# Autodesk Inventor assembly: Maquete Completa_999
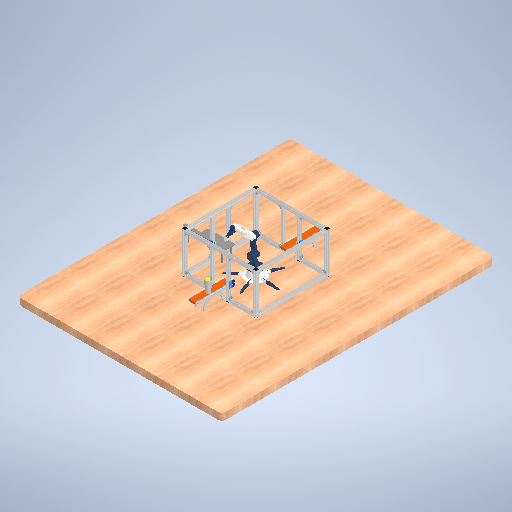
[picture p0: Inventor's stored thumbnail of the model, 512x512]
Saved by Autodesk Inventor 2026 (Build 300175000, 175)
## iProperties
Created: 2024-04-02
Part Number: Maquete Completa_999
Document SubType Name: Assembly
Designer: Gustavo Sousa
Sending System: Autodesk Translation Framework v12.20.1.177
Preprocessor: ST-DEVELOPER v20
Title: Brazo Robtivo 2023 v144.step
## Documents named in this file (40)
- C:\Users\carlo\Documents\Projeto - Braco Robotico\Design\Maquete Completa\Maquete Completa_999.iam
- C:\Users\carlo\Documents\Projeto - Braco Robotico\Design\Maquete Completa\Brazo Robótivo 2023 v144\Engranaje1.ipt
- C:\Users\carlo\Documents\Projeto - Braco Robotico\Design\Maquete Completa\Brazo Robótivo 2023 v144\Engranaje2.ipt
- C:\Users\carlo\Documents\Projeto - Braco Robotico\Design\Maquete Completa\Brazo Robótivo 2023 v144\Barra2.ipt
- C:\Users\carlo\Documents\Projeto - Braco Robotico\Design\Maquete Completa\Brazo Robótivo 2023 v144\Barra1.ipt
- C:\Users\carlo\Documents\Projeto - Braco Robotico\Design\Maquete Completa\Brazo Robótivo 2023 v144\Pinza1.ipt
- C:\Users\carlo\Documents\Projeto - Braco Robotico\Design\Maquete Completa\Brazo Robótivo 2023 v144\Pinza2.ipt
- C:\Users\carlo\Documents\Projeto - Braco Robotico\Design\Maquete Completa\Brazo Robótivo 2023 v144\Base de la garra.ipt
- C:\Users\carlo\Documents\Projeto - Braco Robotico\Design\Maquete Completa\Brazo Robótivo 2023 v144\Base (1) (1).ipt
- C:\Users\carlo\Documents\Projeto - Braco Robotico\Design\Maquete Completa\Brazo Robótivo 2023 v144\Antebrazo (4).ipt
- C:\Users\carlo\Documents\Projeto - Braco Robotico\Design\Maquete Completa\Brazo Robótivo 2023 v144\Muñeca.ipt
- C:\Users\carlo\Documents\Projeto - Braco Robotico\Design\Maquete Completa\Brazo Robótivo 2023 v144\Eje Central.ipt
- C:\Users\carlo\Documents\Projeto - Braco Robotico\Design\Maquete Completa\Brazo Robótivo 2023 v144\Tapa Eje.ipt
- C:\Users\carlo\Documents\Projeto - Braco Robotico\Design\Maquete Completa\Brazo Robótivo 2023 v144\Tapa Base.ipt
- C:\Users\carlo\Documents\Projeto - Braco Robotico\Design\Maquete Completa\Brazo Robótivo 2023 v144\Brazo.ipt
- C:\Users\carlo\Documents\Projeto - Braco Robotico\Design\Maquete Completa\Brazo Robótivo 2023 v144\Tapa garra.ipt
- C:\Users\carlo\Documents\Projeto - Braco Robotico\Design\Maquete Completa\Brazo Robótivo 2023 v144\Pata1.ipt
- C:\Users\carlo\Documents\Projeto - Braco Robotico\Design\Maquete Completa\Brazo Robótivo 2023 v144\Pata2.ipt
- C:\Users\carlo\Documents\Projeto - Braco Robotico\Design\Maquete Completa\Brazo Robótivo 2023 v144\Pata3.ipt
- C:\Users\carlo\Documents\Projeto - Braco Robotico\Design\Maquete Completa\Brazo Robótivo 2023 v144\Pata4.ipt
- C:\Users\carlo\Documents\Projeto - Braco Robotico\Design\Maquete Completa\Brazo Robótivo 2023 v144\Pata5.ipt
- C:\Users\carlo\Documents\Projeto - Braco Robotico\Design\Maquete Completa\Brazo Robótivo 2023 v144\Seguro de servomotor.ipt
- C:\Users\carlo\Documents\Projeto - Braco Robotico\Design\Maquete Completa\maquete_001_001.ipt
- C:\Users\carlo\Documents\Projeto - Braco Robotico\Design\Maquete Completa\perfil_20x20_001.ipt
- C:\Users\carlo\Documents\Projeto - Braco Robotico\Design\Maquete Completa\perfil_20x20_002.ipt
- C:\Users\carlo\Documents\Projeto - Braco Robotico\Design\Maquete Completa\perfil_20x20_003.ipt
- C:\Users\carlo\Documents\Projeto - Braco Robotico\Design\Maquete Completa\perfil_20x20_004.ipt
- C:\Users\carlo\Documents\Projeto - Braco Robotico\Design\Maquete Completa\tampa_001_001.ipt
- C:\Users\carlo\Documents\Projeto - Braco Robotico\Design\Maquete Completa\BPN06M4\BPN06M4\BPN06M4.ipt
- C:\Users\carlo\Documents\Projeto - Braco Robotico\Design\Maquete Completa\CBR2020\CBR2020\CBR2020.ipt
- C:\Users\carlo\Documents\Inventor\Content Center Files\R2026\en-US\BS 4183(4)\BS 4183 - M4 x 8(1) III.ipt
- C:\Users\carlo\Documents\Projeto - Braco Robotico\Design\Maquete Completa\Conveyor_001_001.ipt
- C:\Users\carlo\Documents\Projeto - Braco Robotico\Design\Maquete Completa\Conveyor_002_001.ipt
- C:\Users\carlo\Documents\Projeto - Braco Robotico\Design\Maquete Completa\Conveyor_003_001.ipt
- C:\Users\carlo\Documents\Projeto - Braco Robotico\Design\Maquete Completa\HCSR04 Ultrasonic Sensor\HCSR04 Ultrasonic Sensor\HCSR04 Ultrasonic Sensor.ipt
- C:\Users\carlo\Documents\Projeto - Braco Robotico\Design\Maquete Completa\suporte_ultrassonico_001.ipt
- C:\Users\carlo\Documents\Inventor\Content Center Files\R2026\en-US\BS 4183(1)\BS 4183 - M1,6(1).ipt
- C:\Users\carlo\Documents\Inventor\Content Center Files\R2026\en-US\CSN 02 1131  A\CSN 02 1131 - M1,6 x 6A.ipt
- C:\Users\carlo\Documents\Projeto - Braco Robotico\Design\Maquete Completa\mesa_001.ipt
- C:\Users\carlo\Documents\Projeto - Braco Robotico\Design\Maquete Completa\copo_001.ipt
## Components (249 placed, 39 different names)
1. maquete_001_001:1 — Flush:4, Flush:5, Mate:28, Flush:8, Flush:25, Mate:73, Mate:92, Flush:66, Mate:102, Flush:68, Mate:115, Flush:79, Mate:165
2. mesa_001:1 — Flush:79, Mate:165, Mate:166
3. copo_001:1
4. Engranaje1:1 — Mate:24, Mate:25, Insert:10
5. Engranaje2:1 — Mate:22, Mate:23, Insert:11
6. Barra2:1 — Insert:8, Mate:27
7. Barra1:1 — Insert:9, Mate:26
8. Pinza1:1 — Insert:10, Mate:26
9. Pinza2:1 — Insert:11, Mate:27
10. Base de la garra:1 — Insert:6, Mate:21, Insert:8, Insert:9, Insert:12
11. Base (1) (1):1 — Mate:7, Mate:8, Mate:9, Mate:10, Mate:11, Mate:12, Mate:13, Mate:14, Mate:15, Mate:16, Mate:17, Mate:18, Insert:1, Flush:1, Flush:2, Flush:3, Flush:4, Mate:28
12. Antebrazo (4):1 — Insert:2, Insert:4
13. Muñeca:1 — Insert:5, Insert:12
14. Eje Central:1 — Insert:1, Mate:19, Mate:20, Insert:2
15. Tapa Eje:1 — Mate:19, Mate:20
16. Tapa Base:1 — Mate:17, Mate:18
17. Brazo:1 — Insert:3, Insert:4, Insert:5
18. Tapa garra:1 — Insert:6, Mate:21, Mate:22, Mate:23, Mate:24, Mate:25
19. Pata1:1 — Mate:9, Mate:10
20. Pata2:1 — Mate:11, Mate:12
21. Pata3:1 — Mate:15, Mate:16
22. Pata4:1 — Mate:13, Mate:14
23. Pata5:1 — Mate:7, Mate:8
24. Seguro de servomotor:1 — Insert:3
25. perfil_20x20_001:4 — Flush:6, Mate:29, Flush:7, Flush:8, Flush:9, Mate:30, Flush:10, Flush:29, Flush:62, Mate:75, Flush:63, Flush:65, Mate:77
26. perfil_20x20_002:4 — Flush:6, Mate:29, Flush:7, Flush:11, Flush:26, Flush:27, Mate:37, Flush:28, Mate:49, Flush:51, Flush:52, Mate:50, Mate:67, Flush:60, Mate:68, Mate:74, Mate:76
27. perfil_20x20_002:5 — Flush:9, Mate:30, Flush:10, Mate:31, Flush:12, Flush:13, Mate:32, Flush:14, Flush:15, Mate:33, Flush:16, Mate:47, Flush:49, Mate:48, Mate:61, Flush:58, Mate:62
28. perfil_20x20_001:5 — Flush:11, Mate:31, Flush:12, Symmetry:3, Mate:41, Flush:49, Flush:50, Flush:51
29. perfil_20x20_001:6 — Flush:13, Mate:32, Flush:14, Flush:19, Mate:35, Flush:20, Flush:25, Flush:39, Flush:74
30. perfil_20x20_003:1 — Flush:15, Mate:33, Flush:16, Flush:17, Mate:34, Flush:18, Flush:30
31. perfil_20x20_004:1 — Flush:17, Mate:34, Flush:18, Flush:24, Symmetry:1, Mate:63, Flush:59, Mate:64, Flush:73, Mate:127, Mate:128, Mate:129
32. perfil_20x20_002:6 — Flush:19, Mate:35, Flush:20, Flush:21, Flush:22, Mate:36, Flush:40, Mate:42, Mate:45, Flush:48, Mate:46, Mate:53, Flush:54, Mate:54
33. perfil_20x20_003:2 — Flush:21, Flush:22, Mate:36, Flush:23, Flush:41
34. perfil_20x20_004:2 — Flush:23, Flush:24, Symmetry:1, Flush:42, Mate:65, Mate:66
35. perfil_20x20_001:7 — Flush:26, Flush:27, Mate:37, Flush:33, Mate:39, Flush:34
36. perfil_20x20_003:3 — Flush:28, Flush:29, Flush:30, Flush:31, Flush:32, Mate:38
37. perfil_20x20_004:3 — Flush:31, Flush:32, Mate:38, Symmetry:2, Flush:38, Mate:71, Flush:61, Mate:72, Flush:70, Mate:106, Flush:71, Mate:107, Mate:110
38. perfil_20x20_002:7 — Flush:33, Mate:39, Flush:34, Flush:35, Mate:40, Flush:36, Flush:44, Mate:44, Flush:45, Mate:51, Flush:53, Mate:52, Mate:59, Flush:57, Mate:60, Flush:76, Flush:77
39. perfil_20x20_003:4 — Flush:35, Mate:40, Flush:36, Flush:37
40. perfil_20x20_004:4 — Flush:37, Symmetry:2, Flush:38, Mate:69, Mate:70
41. perfil_20x20_001:8 — Flush:39, Symmetry:3, Mate:41
42. perfil_20x20_003:5 — Flush:40, Flush:41, Mate:42, Mate:43, Flush:43, Symmetry:4
43. perfil_20x20_004:5 — Flush:42, Mate:43, Flush:43, Flush:47, Symmetry:5, Mate:55, Flush:55, Mate:56
44. perfil_20x20_003:6 — Symmetry:4, Flush:44, Mate:44, Flush:45, Flush:46
45. perfil_20x20_004:6 — Flush:46, Flush:47, Symmetry:5, Mate:57, Flush:56, Mate:58, Mate:140, Mate:141, Mate:142, Mate:166
46. tampa_001_001:1 — Mate:45, Flush:48, Mate:46
47. tampa_001_001:2 — Mate:47, Flush:50, Mate:48
48. tampa_001_001:3 — Mate:49, Flush:52, Mate:50
49. tampa_001_001:4 — Mate:51, Flush:53, Mate:52
50. tampa_001_001:5 — Mate:53, Flush:54, Mate:54
51. tampa_001_001:6 — Mate:55, Flush:55, Mate:56
52. tampa_001_001:7 — Mate:57, Flush:56, Mate:58
53. tampa_001_001:8 — Mate:59, Flush:57, Mate:60
54. tampa_001_001:9 — Mate:61, Flush:58, Mate:62
55. tampa_001_001:10 — Mate:67, Flush:60, Mate:68
56. tampa_001_001:11 — Mate:65, Mate:66
57. tampa_001_001:12 — Mate:63, Flush:59, Mate:64
58. tampa_001_001:13 — Mate:71, Flush:61, Mate:72, Mate:73
59. tampa_001_001:14 — Mate:69, Mate:70
60. CBR2020:2
61. BPN06M4:63
62. BPN06M4:64
63. BS 4183 Specification for machine screws and machine screw nuts. Metric series - Metric M4 x 8:63
64. BS 4183 Specification for machine screws and machine screw nuts. Metric series - Metric M4 x 8:64
65. CBR2020:14
66. BPN06M4:87
67. BPN06M4:88
68. BS 4183 Specification for machine screws and machine screw nuts. Metric series - Metric M4 x 8:87
69. BS 4183 Specification for machine screws and machine screw nuts. Metric series - Metric M4 x 8:88
70. CBR2020:15
71. BPN06M4:89
72. BPN06M4:90
73. BS 4183 Specification for machine screws and machine screw nuts. Metric series - Metric M4 x 8:89
74. BS 4183 Specification for machine screws and machine screw nuts. Metric series - Metric M4 x 8:90
75. CBR2020:16
76. BPN06M4:91
77. BPN06M4:92
78. BS 4183 Specification for machine screws and machine screw nuts. Metric series - Metric M4 x 8:91
79. BS 4183 Specification for machine screws and machine screw nuts. Metric series - Metric M4 x 8:92
80. CBR2020:17
81. BPN06M4:93
82. BPN06M4:94
83. BS 4183 Specification for machine screws and machine screw nuts. Metric series - Metric M4 x 8:93
84. BS 4183 Specification for machine screws and machine screw nuts. Metric series - Metric M4 x 8:94
85. CBR2020:18
86. BPN06M4:95
87. BPN06M4:96
88. BS 4183 Specification for machine screws and machine screw nuts. Metric series - Metric M4 x 8:95
89. BS 4183 Specification for machine screws and machine screw nuts. Metric series - Metric M4 x 8:96
90. CBR2020:19
91. BPN06M4:97
92. BPN06M4:98
93. BS 4183 Specification for machine screws and machine screw nuts. Metric series - Metric M4 x 8:97
94. BS 4183 Specification for machine screws and machine screw nuts. Metric series - Metric M4 x 8:98
95. CBR2020:20
96. BPN06M4:99
97. BPN06M4:100
98. BS 4183 Specification for machine screws and machine screw nuts. Metric series - Metric M4 x 8:99
99. BS 4183 Specification for machine screws and machine screw nuts. Metric series - Metric M4 x 8:100
100. CBR2020:21
101. BPN06M4:101
102. BPN06M4:102
103. BS 4183 Specification for machine screws and machine screw nuts. Metric series - Metric M4 x 8:101
104. BS 4183 Specification for machine screws and machine screw nuts. Metric series - Metric M4 x 8:102
105. CBR2020:22
106. BPN06M4:103
107. BPN06M4:104
108. BS 4183 Specification for machine screws and machine screw nuts. Metric series - Metric M4 x 8:103
109. BS 4183 Specification for machine screws and machine screw nuts. Metric series - Metric M4 x 8:104
110. CBR2020:23
111. BPN06M4:105
112. BPN06M4:106
113. BS 4183 Specification for machine screws and machine screw nuts. Metric series - Metric M4 x 8:105
114. BS 4183 Specification for machine screws and machine screw nuts. Metric series - Metric M4 x 8:106
115. CBR2020:24
116. BPN06M4:107
117. BPN06M4:108
118. BS 4183 Specification for machine screws and machine screw nuts. Metric series - Metric M4 x 8:107
119. BS 4183 Specification for machine screws and machine screw nuts. Metric series - Metric M4 x 8:108
120. CBR2020:25
121. BPN06M4:109
122. BPN06M4:110
123. BS 4183 Specification for machine screws and machine screw nuts. Metric series - Metric M4 x 8:109
124. BS 4183 Specification for machine screws and machine screw nuts. Metric series - Metric M4 x 8:110
125. CBR2020:26
126. BPN06M4:111
127. BPN06M4:112
128. BS 4183 Specification for machine screws and machine screw nuts. Metric series - Metric M4 x 8:111
129. BS 4183 Specification for machine screws and machine screw nuts. Metric series - Metric M4 x 8:112
130. CBR2020:27
131. BPN06M4:113
132. BPN06M4:114
133. BS 4183 Specification for machine screws and machine screw nuts. Metric series - Metric M4 x 8:113
134. BS 4183 Specification for machine screws and machine screw nuts. Metric series - Metric M4 x 8:114
135. CBR2020:28
136. BPN06M4:115
137. BPN06M4:116
138. BS 4183 Specification for machine screws and machine screw nuts. Metric series - Metric M4 x 8:115
139. BS 4183 Specification for machine screws and machine screw nuts. Metric series - Metric M4 x 8:116
140. CBR2020:3
141. BPN06M4:65
142. BPN06M4:66
143. BS 4183 Specification for machine screws and machine screw nuts. Metric series - Metric M4 x 8:65
144. BS 4183 Specification for machine screws and machine screw nuts. Metric series - Metric M4 x 8:66
145. CBR2020:4
146. BPN06M4:67
147. BPN06M4:68
148. BS 4183 Specification for machine screws and machine screw nuts. Metric series - Metric M4 x 8:67
149. BS 4183 Specification for machine screws and machine screw nuts. Metric series - Metric M4 x 8:68
150. CBR2020:5
151. BPN06M4:69
152. BPN06M4:70
153. BS 4183 Specification for machine screws and machine screw nuts. Metric series - Metric M4 x 8:69
154. BS 4183 Specification for machine screws and machine screw nuts. Metric series - Metric M4 x 8:70
155. CBR2020:6
156. BPN06M4:71
157. BPN06M4:72
158. BS 4183 Specification for machine screws and machine screw nuts. Metric series - Metric M4 x 8:71
159. BS 4183 Specification for machine screws and machine screw nuts. Metric series - Metric M4 x 8:72
160. CBR2020:7
161. BPN06M4:73
162. BPN06M4:74
163. BS 4183 Specification for machine screws and machine screw nuts. Metric series - Metric M4 x 8:73
164. BS 4183 Specification for machine screws and machine screw nuts. Metric series - Metric M4 x 8:74
165. CBR2020:8
166. BPN06M4:75
167. BPN06M4:76
168. BS 4183 Specification for machine screws and machine screw nuts. Metric series - Metric M4 x 8:75
169. BS 4183 Specification for machine screws and machine screw nuts. Metric series - Metric M4 x 8:76
170. CBR2020:9
171. BPN06M4:77
172. BPN06M4:78
173. BS 4183 Specification for machine screws and machine screw nuts. Metric series - Metric M4 x 8:77
174. BS 4183 Specification for machine screws and machine screw nuts. Metric series - Metric M4 x 8:78
175. CBR2020:10
176. BPN06M4:79
177. BPN06M4:80
178. BS 4183 Specification for machine screws and machine screw nuts. Metric series - Metric M4 x 8:79
179. BS 4183 Specification for machine screws and machine screw nuts. Metric series - Metric M4 x 8:80
180. CBR2020:11
181. BPN06M4:81
182. BPN06M4:82
183. BS 4183 Specification for machine screws and machine screw nuts. Metric series - Metric M4 x 8:81
184. BS 4183 Specification for machine screws and machine screw nuts. Metric series - Metric M4 x 8:82
185. CBR2020:12
186. BPN06M4:83
187. BPN06M4:84
188. BS 4183 Specification for machine screws and machine screw nuts. Metric series - Metric M4 x 8:83
189. BS 4183 Specification for machine screws and machine screw nuts. Metric series - Metric M4 x 8:84
190. CBR2020:13
191. BPN06M4:85
192. BPN06M4:86
193. BS 4183 Specification for machine screws and machine screw nuts. Metric series - Metric M4 x 8:85
194. BS 4183 Specification for machine screws and machine screw nuts. Metric series - Metric M4 x 8:86
195. CBR2020:1 — Flush:62, Mate:74, Mate:75, Flush:64, Mate:78, Mate:80, Mate:82
196. BPN06M4:1 — Flush:65, Mate:77, Mate:78, Mate:81
197. BPN06M4:2 — Flush:63, Mate:76, Flush:64, Mate:79
198. BS 4183 Specification for machine screws and machine screw nuts. Metric series - Metric M4 x 8:1 — Mate:79, Mate:80
199. BS 4183 Specification for machine screws and machine screw nuts. Metric series - Metric M4 x 8:2 — Mate:81, Mate:82
200. Conveyor_002_001:1 — Mate:83, Mate:84, Mate:85, Mate:91
201. Conveyor_002_001:2 — Mate:86, Mate:87, Mate:88, Mate:89
202. Conveyor_003_001:1 — Mate:89, Mate:90, Mate:91
203. Conveyor_001_001:2 — Mate:83, Mate:84, Mate:85, Mate:86, Mate:87, Mate:88, Mate:90, Mate:92, Flush:66, Flush:72
204. Conveyor_001_001:3 — Mate:102, Flush:68, Flush:75
205. Conveyor_002_001:3
206. Conveyor_002_001:4
207. Conveyor_003_001:2
208. suporte_ultrassonico_001:3 — Mate:137, Mate:138, Mate:139, Mate:142, Mate:143, Mate:144, Mate:145, Mate:146, Mate:147, Mate:148, Mate:149, Mate:150, Mate:151, Mate:152, Mate:153, Mate:154, Mate:155, Mate:156
209. HCSR04 Ultrasonic Sensor:3 — Mate:137, Mate:138, Mate:139, Flush:78, Mate:161, Mate:162, Mate:163, Mate:164
210. BPN06M4:61 — Flush:77, Mate:141, Mate:144
211. BPN06M4:62 — Flush:76, Mate:140, Mate:143
212. BS 4183 Specification for machine screws and machine screw nuts. Metric series - Metric M4 x 8:61 — Mate:145, Mate:147
213. BS 4183 Specification for machine screws and machine screw nuts. Metric series - Metric M4 x 8:62 — Mate:146, Mate:148
214. CSN 02 1131 A M1,6 x 6:9 — Mate:149, Mate:154, Mate:157
215. CSN 02 1131 A M1,6 x 6:10 — Mate:152, Mate:156, Mate:160
216. CSN 02 1131 A M1,6 x 6:11 — Mate:151, Mate:155, Mate:159
217. CSN 02 1131 A M1,6 x 6:12 — Mate:150, Mate:153, Mate:158
218. BS 4183 - Metric M1,6:9 — Mate:158, Mate:162
219. BS 4183 - Metric M1,6:10 — Mate:160, Mate:163
220. BS 4183 - Metric M1,6:11 — Mate:159, Mate:164
221. BS 4183 - Metric M1,6:12 — Mate:157, Mate:161
222. suporte_ultrassonico_001:2 — Mate:116, Mate:117, Mate:118, Insert:21, Insert:22, Insert:23, Insert:24, Mate:129, Mate:130, Mate:131, Mate:132, Mate:133, Mate:134, Mate:135
223. HCSR04 Ultrasonic Sensor:2 — Mate:116, Mate:117, Mate:118, Mate:120, Mate:122, Mate:124, Mate:126, Mate:136, Flush:75
224. CSN 02 1131 A M1,6 x 6:5 — Insert:21, Mate:123
225. CSN 02 1131 A M1,6 x 6:6 — Insert:22, Mate:125
226. CSN 02 1131 A M1,6 x 6:7 — Insert:23, Mate:119
227. CSN 02 1131 A M1,6 x 6:8 — Insert:24, Mate:121
228. BS 4183 - Metric M1,6:5 — Mate:119, Mate:120
229. BS 4183 - Metric M1,6:6 — Mate:121, Mate:122
230. BS 4183 - Metric M1,6:7 — Mate:123, Mate:124
231. BS 4183 - Metric M1,6:8 — Mate:125, Mate:126
232. BPN06M4:59 — Flush:74, Mate:128, Mate:131
233. BPN06M4:60 — Flush:73, Mate:127, Mate:130
234. BS 4183 Specification for machine screws and machine screw nuts. Metric series - Metric M4 x 8:59 — Mate:133, Mate:134
235. BS 4183 Specification for machine screws and machine screw nuts. Metric series - Metric M4 x 8:60 — Mate:132, Mate:135
236. BS 4183 - Metric M1,6:1 — Insert:13
237. BS 4183 - Metric M1,6:2 — Insert:14
238. BS 4183 - Metric M1,6:3 — Insert:15
239. BS 4183 - Metric M1,6:4 — Insert:16
240. CSN 02 1131 A M1,6 x 6:2 — Insert:17
241. CSN 02 1131 A M1,6 x 6:3 — Insert:18
242. CSN 02 1131 A M1,6 x 6:1 — Insert:19
243. CSN 02 1131 A M1,6 x 6:4 — Insert:20
244. HCSR04 Ultrasonic Sensor:1 — Mate:103, Mate:104, Mate:105, Insert:13, Insert:14, Insert:15, Insert:16, Flush:72, Mate:136, Flush:78
245. suporte_ultrassonico_001:1 — Mate:103, Mate:104, Mate:105, Mate:108, Mate:109, Mate:110, Mate:112, Mate:114, Mate:115, Insert:17, Insert:18, Insert:19, Insert:20
246. BPN06M4:58 — Flush:70, Mate:106, Mate:109, Mate:111
247. BS 4183 Specification for machine screws and machine screw nuts. Metric series - Metric M4 x 8:57 — Mate:111, Mate:112
248. BS 4183 Specification for machine screws and machine screw nuts. Metric series - Metric M4 x 8:58 — Mate:113, Mate:114
249. BPN06M4:57 — Flush:71, Mate:107, Mate:108, Mate:113
## Relationships (265: Mate 160, Flush 77, Insert 23, Symmetry 5)
- Mate:7: Base (1) (1):1 ↔ Pata5:1
- Mate:8: Base (1) (1):1 ↔ Pata5:1
- Mate:9: Base (1) (1):1 ↔ Pata1:1
- Mate:10: Base (1) (1):1 ↔ Pata1:1
- Mate:11: Base (1) (1):1 ↔ Pata2:1
- Mate:12: Base (1) (1):1 ↔ Pata2:1
- Mate:13: Base (1) (1):1 ↔ Pata4:1
- Mate:14: Base (1) (1):1 ↔ Pata4:1
- Mate:15: Base (1) (1):1 ↔ Pata3:1
- Mate:16: Base (1) (1):1 ↔ Pata3:1
- Mate:17: Base (1) (1):1 ↔ Tapa Base:1
- Mate:18: Base (1) (1):1 ↔ Tapa Base:1
- Insert:1: Base (1) (1):1 ↔ Eje Central:1
- Mate:19: Eje Central:1 ↔ Tapa Eje:1
- Mate:20 (1.05 mm): Eje Central:1 ↔ Tapa Eje:1
- Insert:2: Antebrazo (4):1 ↔ Eje Central:1
- Insert:3: Brazo:1 ↔ Seguro de servomotor:1
- Insert:4: Antebrazo (4):1 ↔ Brazo:1
- Insert:5: Muñeca:1 ↔ Brazo:1
- Insert:6: Base de la garra:1 ↔ Tapa garra:1
- Mate:21: Base de la garra:1 ↔ Tapa garra:1
- Insert:8: Barra2:1 ↔ Base de la garra:1
- Insert:9: Barra1:1 ↔ Base de la garra:1
- Mate:22: Engranaje2:1 ↔ Tapa garra:1
- Mate:23: Engranaje2:1 ↔ Tapa garra:1
- Mate:24: Engranaje1:1 ↔ Tapa garra:1
- Mate:25: Engranaje1:1 ↔ Tapa garra:1
- Insert:10 (0.5 mm): Engranaje1:1 ↔ Pinza1:1
- Mate:26: Barra1:1 ↔ Pinza1:1
- Insert:11: Engranaje2:1 ↔ Pinza2:1
- Mate:27: Barra2:1 ↔ Pinza2:1
- Insert:12: Base de la garra:1 ↔ Muñeca:1
- Flush:1: Base (1) (1):1
- Flush:2: Base (1) (1):1
- Flush:3: Base (1) (1):1
- Flush:4: maquete_001_001:1 ↔ Base (1) (1):1
- Flush:5: maquete_001_001:1
- Mate:28: maquete_001_001:1 ↔ Base (1) (1):1
- Flush:6: perfil_20x20_001:4 ↔ perfil_20x20_002:4
- Mate:29: perfil_20x20_001:4 ↔ perfil_20x20_002:4
- Flush:7: perfil_20x20_001:4 ↔ perfil_20x20_002:4
- Flush:8: maquete_001_001:1 ↔ perfil_20x20_001:4
- Flush:9: perfil_20x20_001:4 ↔ perfil_20x20_002:5
- Mate:30: perfil_20x20_001:4 ↔ perfil_20x20_002:5
- Flush:10: perfil_20x20_001:4 ↔ perfil_20x20_002:5
- Flush:11: perfil_20x20_002:4 ↔ perfil_20x20_001:5
- Mate:31: perfil_20x20_002:5 ↔ perfil_20x20_001:5
- Flush:12: perfil_20x20_002:5 ↔ perfil_20x20_001:5
- Flush:13: perfil_20x20_002:5 ↔ perfil_20x20_001:6
- Mate:32: perfil_20x20_002:5 ↔ perfil_20x20_001:6
- Flush:14: perfil_20x20_002:5 ↔ perfil_20x20_001:6
- Flush:15: perfil_20x20_002:5 ↔ perfil_20x20_003:1
- Mate:33: perfil_20x20_002:5 ↔ perfil_20x20_003:1
- Flush:16: perfil_20x20_002:5 ↔ perfil_20x20_003:1
- Flush:17: perfil_20x20_003:1 ↔ perfil_20x20_004:1
- Mate:34: perfil_20x20_003:1 ↔ perfil_20x20_004:1
- Flush:18: perfil_20x20_003:1 ↔ perfil_20x20_004:1
- Flush:19: perfil_20x20_001:6 ↔ perfil_20x20_002:6
- Mate:35: perfil_20x20_001:6 ↔ perfil_20x20_002:6
- Flush:20: perfil_20x20_001:6 ↔ perfil_20x20_002:6
- Flush:21: perfil_20x20_002:6 ↔ perfil_20x20_003:2
- Flush:22: perfil_20x20_002:6 ↔ perfil_20x20_003:2
- Mate:36: perfil_20x20_002:6 ↔ perfil_20x20_003:2
- Flush:23: perfil_20x20_003:2 ↔ perfil_20x20_004:2
- Flush:24: perfil_20x20_004:1 ↔ perfil_20x20_004:2
- Symmetry:1: perfil_20x20_004:1 ↔ perfil_20x20_004:2
- Flush:25: maquete_001_001:1 ↔ perfil_20x20_001:6
- Flush:26: perfil_20x20_002:4 ↔ perfil_20x20_001:7
- Flush:27: perfil_20x20_002:4 ↔ perfil_20x20_001:7
- Mate:37: perfil_20x20_002:4 ↔ perfil_20x20_001:7
- Flush:28: perfil_20x20_002:4 ↔ perfil_20x20_003:3
- Flush:29: perfil_20x20_001:4 ↔ perfil_20x20_003:3
- Flush:30: perfil_20x20_003:1 ↔ perfil_20x20_003:3
- Flush:31: perfil_20x20_003:3 ↔ perfil_20x20_004:3
- Flush:32: perfil_20x20_003:3 ↔ perfil_20x20_004:3
- Mate:38: perfil_20x20_003:3 ↔ perfil_20x20_004:3
- Flush:33: perfil_20x20_001:7 ↔ perfil_20x20_002:7
- Mate:39: perfil_20x20_001:7 ↔ perfil_20x20_002:7
- Flush:34: perfil_20x20_001:7 ↔ perfil_20x20_002:7
- Flush:35: perfil_20x20_002:7 ↔ perfil_20x20_003:4
- Mate:40: perfil_20x20_002:7 ↔ perfil_20x20_003:4
- Flush:36: perfil_20x20_002:7 ↔ perfil_20x20_003:4
- Flush:37: perfil_20x20_003:4 ↔ perfil_20x20_004:4
- Symmetry:2: perfil_20x20_004:3 ↔ perfil_20x20_004:4
- Flush:38: perfil_20x20_004:3 ↔ perfil_20x20_004:4
- Flush:39: perfil_20x20_001:6 ↔ perfil_20x20_001:8
- Symmetry:3: perfil_20x20_001:5 ↔ perfil_20x20_001:8
- Mate:41: perfil_20x20_001:5 ↔ perfil_20x20_001:8
- Flush:40: perfil_20x20_002:6 ↔ perfil_20x20_003:5
- Flush:41: perfil_20x20_003:2 ↔ perfil_20x20_003:5
- Mate:42: perfil_20x20_002:6 ↔ perfil_20x20_003:5
- Flush:42: perfil_20x20_004:2 ↔ perfil_20x20_004:5
- Mate:43: perfil_20x20_003:5 ↔ perfil_20x20_004:5
- Flush:43: perfil_20x20_003:5 ↔ perfil_20x20_004:5
- Symmetry:4: perfil_20x20_003:5 ↔ perfil_20x20_003:6
- Flush:44: perfil_20x20_002:7 ↔ perfil_20x20_003:6
- Mate:44: perfil_20x20_002:7 ↔ perfil_20x20_003:6
- Flush:45: perfil_20x20_002:7 ↔ perfil_20x20_003:6
- Flush:46: perfil_20x20_003:6 ↔ perfil_20x20_004:6
- Flush:47: perfil_20x20_004:5 ↔ perfil_20x20_004:6
- Symmetry:5: perfil_20x20_004:5 ↔ perfil_20x20_004:6
- Mate:45: perfil_20x20_002:6 ↔ tampa_001_001:1
- Flush:48: perfil_20x20_002:6 ↔ tampa_001_001:1
- Mate:46: perfil_20x20_002:6 ↔ tampa_001_001:1
- Mate:47: perfil_20x20_002:5 ↔ tampa_001_001:2
- Flush:49: perfil_20x20_002:5 ↔ perfil_20x20_001:5
- Flush:50: perfil_20x20_001:5 ↔ tampa_001_001:2
- Mate:48: perfil_20x20_002:5 ↔ tampa_001_001:2
- Mate:49: perfil_20x20_002:4 ↔ tampa_001_001:3
- Flush:51: perfil_20x20_002:4 ↔ perfil_20x20_001:5
- Flush:52: perfil_20x20_002:4 ↔ tampa_001_001:3
- Mate:50: perfil_20x20_002:4 ↔ tampa_001_001:3
- Mate:51: perfil_20x20_002:7 ↔ tampa_001_001:4
- Flush:53: perfil_20x20_002:7 ↔ tampa_001_001:4
- Mate:52: perfil_20x20_002:7 ↔ tampa_001_001:4
- Mate:53: perfil_20x20_002:6 ↔ tampa_001_001:5
- Flush:54: perfil_20x20_002:6 ↔ tampa_001_001:5
- Mate:54: perfil_20x20_002:6 ↔ tampa_001_001:5
- Mate:55: perfil_20x20_004:5 ↔ tampa_001_001:6
- Flush:55: perfil_20x20_004:5 ↔ tampa_001_001:6
- Mate:56: perfil_20x20_004:5 ↔ tampa_001_001:6
- Mate:57: perfil_20x20_004:6 ↔ tampa_001_001:7
- Flush:56: perfil_20x20_004:6 ↔ tampa_001_001:7
- Mate:58: perfil_20x20_004:6 ↔ tampa_001_001:7
- Mate:59: perfil_20x20_002:7 ↔ tampa_001_001:8
- Flush:57: perfil_20x20_002:7 ↔ tampa_001_001:8
- Mate:60: perfil_20x20_002:7 ↔ tampa_001_001:8
- Mate:61: perfil_20x20_002:5 ↔ tampa_001_001:9
- Flush:58: perfil_20x20_002:5 ↔ tampa_001_001:9
- Mate:62: perfil_20x20_002:5 ↔ tampa_001_001:9
- Mate:63: perfil_20x20_004:1 ↔ tampa_001_001:12
- Flush:59: perfil_20x20_004:1 ↔ tampa_001_001:12
- Mate:64: perfil_20x20_004:1 ↔ tampa_001_001:12
- Mate:65: perfil_20x20_004:2 ↔ tampa_001_001:11
- Mate:66: perfil_20x20_004:2 ↔ tampa_001_001:11
- Mate:67: perfil_20x20_002:4 ↔ tampa_001_001:10
- Flush:60: perfil_20x20_002:4 ↔ tampa_001_001:10
- Mate:68: perfil_20x20_002:4 ↔ tampa_001_001:10
- Mate:69: perfil_20x20_004:4 ↔ tampa_001_001:14
- Mate:70: perfil_20x20_004:4 ↔ tampa_001_001:14
- Mate:71: perfil_20x20_004:3 ↔ tampa_001_001:13
- Flush:61: perfil_20x20_004:3 ↔ tampa_001_001:13
- Mate:72: perfil_20x20_004:3 ↔ tampa_001_001:13
- Mate:73: maquete_001_001:1 ↔ tampa_001_001:13
- Flush:62: perfil_20x20_001:4 ↔ CBR2020:1
- Mate:74: perfil_20x20_002:4 ↔ CBR2020:1
- Mate:75: perfil_20x20_001:4 ↔ CBR2020:1
- Flush:63: perfil_20x20_001:4 ↔ BPN06M4:2
- Mate:76: perfil_20x20_002:4 ↔ BPN06M4:2
- Flush:64: CBR2020:1 ↔ BPN06M4:2
- Flush:65: perfil_20x20_001:4 ↔ BPN06M4:1
- Mate:77: perfil_20x20_001:4 ↔ BPN06M4:1
- Mate:78: CBR2020:1 ↔ BPN06M4:1
- Mate:79: BPN06M4:2 ↔ BS 4183 Specification for machine screws and machine screw nuts. Metric series - Metric M4 x 8:1
- Mate:80: CBR2020:1 ↔ BS 4183 Specification for machine screws and machine screw nuts. Metric series - Metric M4 x 8:1
- Mate:81: BPN06M4:1 ↔ BS 4183 Specification for machine screws and machine screw nuts. Metric series - Metric M4 x 8:2
- Mate:82: CBR2020:1 ↔ BS 4183 Specification for machine screws and machine screw nuts. Metric series - Metric M4 x 8:2
- Mate:83: Conveyor_002_001:1 ↔ Conveyor_001_001:2
- Mate:84: Conveyor_002_001:1 ↔ Conveyor_001_001:2
- Mate:85 (1 mm): Conveyor_002_001:1 ↔ Conveyor_001_001:2
- Mate:86: Conveyor_002_001:2 ↔ Conveyor_001_001:2
- Mate:87: Conveyor_002_001:2 ↔ Conveyor_001_001:2
- Mate:88 (1 mm): Conveyor_002_001:2 ↔ Conveyor_001_001:2
- Mate:89: Conveyor_002_001:2 ↔ Conveyor_003_001:1
- Mate:90 (1.5 mm): Conveyor_003_001:1 ↔ Conveyor_001_001:2
- Mate:91: Conveyor_002_001:1 ↔ Conveyor_003_001:1
- Mate:92: maquete_001_001:1 ↔ Conveyor_001_001:2
- Flush:66: maquete_001_001:1 ↔ Conveyor_001_001:2
- [Mate]: Conveyor_001_001:3 ↔ Conveyor_002_001:3
- [Mate]: Conveyor_001_001:3 ↔ Conveyor_002_001:3
- [Mate] (1 mm): Conveyor_001_001:3 ↔ Conveyor_002_001:3
- [Mate]: Conveyor_001_001:3 ↔ Conveyor_002_001:4
- [Mate]: Conveyor_001_001:3 ↔ Conveyor_002_001:4
- [Mate] (1 mm): Conveyor_001_001:3 ↔ Conveyor_002_001:4
- [Mate]: Conveyor_002_001:4 ↔ Conveyor_003_001:2
- [Mate] (1.5 mm): Conveyor_001_001:3 ↔ Conveyor_003_001:2
- [Mate]: Conveyor_002_001:3 ↔ Conveyor_003_001:2
- Mate:102: maquete_001_001:1 ↔ Conveyor_001_001:3
- Flush:68: maquete_001_001:1 ↔ Conveyor_001_001:3
- Mate:103: HCSR04 Ultrasonic Sensor:1 ↔ suporte_ultrassonico_001:1
- Mate:104: HCSR04 Ultrasonic Sensor:1 ↔ suporte_ultrassonico_001:1
- Mate:105: HCSR04 Ultrasonic Sensor:1 ↔ suporte_ultrassonico_001:1
- Flush:70: perfil_20x20_004:3 ↔ BPN06M4:58
- Mate:106: perfil_20x20_004:3 ↔ BPN06M4:58
- Flush:71: perfil_20x20_004:3 ↔ BPN06M4:57
- Mate:107: perfil_20x20_004:3 ↔ BPN06M4:57
- Mate:108: suporte_ultrassonico_001:1 ↔ BPN06M4:57
- Mate:109: suporte_ultrassonico_001:1 ↔ BPN06M4:58
- Mate:110: perfil_20x20_004:3 ↔ suporte_ultrassonico_001:1
- Mate:111: BPN06M4:58 ↔ BS 4183 Specification for machine screws and machine screw nuts. Metric series - Metric M4 x 8:57
- Mate:112: suporte_ultrassonico_001:1 ↔ BS 4183 Specification for machine screws and machine screw nuts. Metric series - Metric M4 x 8:57
- Mate:113: BS 4183 Specification for machine screws and machine screw nuts. Metric series - Metric M4 x 8:58 ↔ BPN06M4:57
- Mate:114: suporte_ultrassonico_001:1 ↔ BS 4183 Specification for machine screws and machine screw nuts. Metric series - Metric M4 x 8:58
- Mate:115 (90 mm): maquete_001_001:1 ↔ suporte_ultrassonico_001:1
- Insert:13: BS 4183 - Metric M1,6:1 ↔ HCSR04 Ultrasonic Sensor:1
- Insert:14: BS 4183 - Metric M1,6:2 ↔ HCSR04 Ultrasonic Sensor:1
- Insert:15: BS 4183 - Metric M1,6:3 ↔ HCSR04 Ultrasonic Sensor:1
- Insert:16: BS 4183 - Metric M1,6:4 ↔ HCSR04 Ultrasonic Sensor:1
- Insert:17: CSN 02 1131 A M1,6 x 6:2 ↔ suporte_ultrassonico_001:1
- Insert:18: CSN 02 1131 A M1,6 x 6:3 ↔ suporte_ultrassonico_001:1
- Insert:19: CSN 02 1131 A M1,6 x 6:1 ↔ suporte_ultrassonico_001:1
- Insert:20: CSN 02 1131 A M1,6 x 6:4 ↔ suporte_ultrassonico_001:1
- Flush:72 (-30 mm): Conveyor_001_001:2 ↔ HCSR04 Ultrasonic Sensor:1
- Mate:116: suporte_ultrassonico_001:2 ↔ HCSR04 Ultrasonic Sensor:2
- Mate:117: suporte_ultrassonico_001:2 ↔ HCSR04 Ultrasonic Sensor:2
- Mate:118: suporte_ultrassonico_001:2 ↔ HCSR04 Ultrasonic Sensor:2
- Insert:21: suporte_ultrassonico_001:2 ↔ CSN 02 1131 A M1,6 x 6:5
- Insert:22: suporte_ultrassonico_001:2 ↔ CSN 02 1131 A M1,6 x 6:6
- Insert:23: suporte_ultrassonico_001:2 ↔ CSN 02 1131 A M1,6 x 6:7
- Insert:24: suporte_ultrassonico_001:2 ↔ CSN 02 1131 A M1,6 x 6:8
- Mate:119: CSN 02 1131 A M1,6 x 6:7 ↔ BS 4183 - Metric M1,6:5
- Mate:120: HCSR04 Ultrasonic Sensor:2 ↔ BS 4183 - Metric M1,6:5
- Mate:121: CSN 02 1131 A M1,6 x 6:8 ↔ BS 4183 - Metric M1,6:6
- Mate:122: HCSR04 Ultrasonic Sensor:2 ↔ BS 4183 - Metric M1,6:6
- Mate:123: CSN 02 1131 A M1,6 x 6:5 ↔ BS 4183 - Metric M1,6:7
- Mate:124: HCSR04 Ultrasonic Sensor:2 ↔ BS 4183 - Metric M1,6:7
- Mate:125: CSN 02 1131 A M1,6 x 6:6 ↔ BS 4183 - Metric M1,6:8
- Mate:126: HCSR04 Ultrasonic Sensor:2 ↔ BS 4183 - Metric M1,6:8
- Flush:73: perfil_20x20_004:1 ↔ BPN06M4:60
- Mate:127: perfil_20x20_004:1 ↔ BPN06M4:60
- Flush:74: perfil_20x20_001:6 ↔ BPN06M4:59
- Mate:128: perfil_20x20_004:1 ↔ BPN06M4:59
- Mate:129: perfil_20x20_004:1 ↔ suporte_ultrassonico_001:2
- Mate:130: suporte_ultrassonico_001:2 ↔ BPN06M4:60
- Mate:131: suporte_ultrassonico_001:2 ↔ BPN06M4:59
- Mate:132: suporte_ultrassonico_001:2 ↔ BS 4183 Specification for machine screws and machine screw nuts. Metric series - Metric M4 x 8:60
- Mate:133: suporte_ultrassonico_001:2 ↔ BS 4183 Specification for machine screws and machine screw nuts. Metric series - Metric M4 x 8:59
- Mate:134: suporte_ultrassonico_001:2 ↔ BS 4183 Specification for machine screws and machine screw nuts. Metric series - Metric M4 x 8:59
- Mate:135: suporte_ultrassonico_001:2 ↔ BS 4183 Specification for machine screws and machine screw nuts. Metric series - Metric M4 x 8:60
- Mate:136: HCSR04 Ultrasonic Sensor:2 ↔ HCSR04 Ultrasonic Sensor:1
- Flush:75 (30 mm): Conveyor_001_001:3 ↔ HCSR04 Ultrasonic Sensor:2
- Mate:137: suporte_ultrassonico_001:3 ↔ HCSR04 Ultrasonic Sensor:3
- Mate:138: suporte_ultrassonico_001:3 ↔ HCSR04 Ultrasonic Sensor:3
- Mate:139: suporte_ultrassonico_001:3 ↔ HCSR04 Ultrasonic Sensor:3
- Flush:76: perfil_20x20_002:7 ↔ BPN06M4:62
- Mate:140: perfil_20x20_004:6 ↔ BPN06M4:62
- Flush:77: perfil_20x20_002:7 ↔ BPN06M4:61
- Mate:141: perfil_20x20_004:6 ↔ BPN06M4:61
- Mate:142: perfil_20x20_004:6 ↔ suporte_ultrassonico_001:3
- Mate:143: suporte_ultrassonico_001:3 ↔ BPN06M4:62
- Mate:144: suporte_ultrassonico_001:3 ↔ BPN06M4:61
- Mate:145: suporte_ultrassonico_001:3 ↔ BS 4183 Specification for machine screws and machine screw nuts. Metric series - Metric M4 x 8:61
- Mate:146: suporte_ultrassonico_001:3 ↔ BS 4183 Specification for machine screws and machine screw nuts. Metric series - Metric M4 x 8:62
- Mate:147: suporte_ultrassonico_001:3 ↔ BS 4183 Specification for machine screws and machine screw nuts. Metric series - Metric M4 x 8:61
- Mate:148: suporte_ultrassonico_001:3 ↔ BS 4183 Specification for machine screws and machine screw nuts. Metric series - Metric M4 x 8:62
- Flush:78: HCSR04 Ultrasonic Sensor:3 ↔ HCSR04 Ultrasonic Sensor:1
- Mate:149: suporte_ultrassonico_001:3 ↔ CSN 02 1131 A M1,6 x 6:9
- Mate:150: suporte_ultrassonico_001:3 ↔ CSN 02 1131 A M1,6 x 6:12
- Mate:151: suporte_ultrassonico_001:3 ↔ CSN 02 1131 A M1,6 x 6:11
- Mate:152: suporte_ultrassonico_001:3 ↔ CSN 02 1131 A M1,6 x 6:10
- Mate:153: suporte_ultrassonico_001:3 ↔ CSN 02 1131 A M1,6 x 6:12
- Mate:154: suporte_ultrassonico_001:3 ↔ CSN 02 1131 A M1,6 x 6:9
- Mate:155: suporte_ultrassonico_001:3 ↔ CSN 02 1131 A M1,6 x 6:11
- Mate:156: suporte_ultrassonico_001:3 ↔ CSN 02 1131 A M1,6 x 6:10
- Mate:157: CSN 02 1131 A M1,6 x 6:9 ↔ BS 4183 - Metric M1,6:12
- Mate:158: CSN 02 1131 A M1,6 x 6:12 ↔ BS 4183 - Metric M1,6:9
- Mate:159: CSN 02 1131 A M1,6 x 6:11 ↔ BS 4183 - Metric M1,6:11
- Mate:160: CSN 02 1131 A M1,6 x 6:10 ↔ BS 4183 - Metric M1,6:10
- Mate:161: HCSR04 Ultrasonic Sensor:3 ↔ BS 4183 - Metric M1,6:12
- Mate:162: HCSR04 Ultrasonic Sensor:3 ↔ BS 4183 - Metric M1,6:9
- Mate:163: HCSR04 Ultrasonic Sensor:3 ↔ BS 4183 - Metric M1,6:10
- Mate:164: HCSR04 Ultrasonic Sensor:3 ↔ BS 4183 - Metric M1,6:11
- Flush:79: maquete_001_001:1 ↔ mesa_001:1
- Mate:165: maquete_001_001:1 ↔ mesa_001:1
- Mate:166: mesa_001:1 ↔ perfil_20x20_004:6
## Named parameters: d232_d219 = 0 mm, d233_d220 = 0 mm, d234_d221 = 1 mm, d235_d222 = 0 mm, d236_d223 = 0 mm, d237_d224 = 1 mm, d238_d225 = 0 mm, d239_d226 = 1.5 mm, d240_d227 = 0 mm
